# Autodesk Inventor assembly: WheelPulleyAssembly
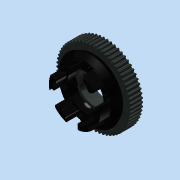
[picture p0: Inventor's stored thumbnail of the model, 180x180]
Saved by Autodesk Inventor 2015 (Build 190159000, 159)
## iProperties
Created: 2015-11-06
Part Number: WheelPulleyAssembly
Document SubType Name: Assembly
Designer: Raphael
Author: Raphael
## Documents named in this file (3)
- \\psf\Home\Documents\electric-skateboard\CAD\WheelPulleyAssembly.iam
- \\psf\Home\Documents\electric-skateboard\CAD\62tPulley.ipt
- \\psf\Home\Documents\electric-skateboard\CAD\WheelInsert.ipt
## Components (2 placed, 2 different names)
1. 62tPulley:1 — Mate:1, Mate:2, Mate:3
2. WheelInsert:1 — Mate:1, Mate:2, Mate:3
## Relationships (3: Mate 3)
- Mate:1: 62tPulley:1 ↔ WheelInsert:1
- Mate:2: 62tPulley:1 ↔ WheelInsert:1
- Mate:3: 62tPulley:1 ↔ WheelInsert:1
